# Autodesk Inventor assembly: Motor Front Assembly
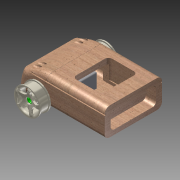
[picture p0: Inventor's stored thumbnail of the model, 180x180]
Saved by Autodesk Inventor 2015 (Build 190159000, 159)
## iProperties
Created: 2018-02-28
Part Number: Motor Front Assembly
Document SubType Name: Assembly
Designer: Administrator
Author: Administrator
## Documents named in this file (9)
- L:\IED 9th\Automoblox\7.4 Exact Parts\Motor Front Assembly.iam
- L:\IED 9th\Automoblox\7.4 Exact Parts\Motor Front.ipt
- L:\IED 9th\Automoblox\7.4 Exact Parts\Motor Gear.ipt
- L:\IED 9th\Automoblox\7.4 Exact Parts\Motor.ipt
- L:\IED 9th\Automoblox\7.4 Exact Parts\Motor Passenger Section.ipt
- L:\IED 9th\Automoblox\7.4 Exact Parts\Motor 9V Battery.ipt
- L:\IED 9th\Automoblox\7.4 Exact Parts\Motor Axle Connection 2.ipt
- L:\IED 9th\Automoblox\7.4 Exact Parts\Motor Axle Connection.ipt
- L:\IED 9th\Automoblox\7.4 Exact Parts\T9 Wheel.ipt
## Components (9 placed, 8 different names)
1. Motor Front:1 — Tangent:1, Tangent:2, Mate:7, Flush:1, Flush:2, Mate:10, Mate:11
2. Motor Gear:1 — Mate:5, Mate:6
3. Motor:1 — Mate:5, Mate:6, Tangent:1, Tangent:2, Tangent:3
4. Motor Passenger Section:1 — Mate:7, Flush:1, Flush:2, Mate:12, Mate:13
5. Motor Axle Connection 2:1 — Mate:8, Mate:9, Insert:1, Mate:11, Insert:2
6. Motor Axle Connection:1 — Mate:8, Mate:9, Insert:1, Mate:10, Insert:3
7. T9 Wheel:1 — Insert:3
8. T9 Wheel:2 — Insert:2
9. Motor 9V Battery:1 — Mate:12, Mate:13, Tangent:3
## Relationships (17: Mate 9, Tangent 3, Insert 3, Flush 2)
- Mate:5: Motor Gear:1 ↔ Motor:1
- Mate:6: Motor Gear:1 ↔ Motor:1
- Tangent:1: Motor Front:1 ↔ Motor:1
- Tangent:2: Motor Front:1 ↔ Motor:1
- Mate:7: Motor Front:1 ↔ Motor Passenger Section:1
- Flush:1: Motor Front:1 ↔ Motor Passenger Section:1
- Flush:2: Motor Front:1 ↔ Motor Passenger Section:1
- Mate:8: Motor Axle Connection 2:1 ↔ Motor Axle Connection:1
- Mate:9: Motor Axle Connection 2:1 ↔ Motor Axle Connection:1
- Insert:1: Motor Axle Connection 2:1 ↔ Motor Axle Connection:1
- Mate:10: Motor Front:1 ↔ Motor Axle Connection:1
- Mate:11: Motor Front:1 ↔ Motor Axle Connection 2:1
- Insert:2: Motor Axle Connection 2:1 ↔ T9 Wheel:2
- Insert:3: Motor Axle Connection:1 ↔ T9 Wheel:1
- Mate:12: Motor Passenger Section:1 ↔ Motor 9V Battery:1
- Mate:13: Motor Passenger Section:1 ↔ Motor 9V Battery:1
- Tangent:3: Motor:1 ↔ Motor 9V Battery:1
